# Autodesk Inventor assembly: Tri_Act_lite
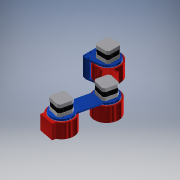
[picture p0: Inventor's stored thumbnail of the model, 180x180]
Saved by Autodesk Inventor 2017 (Build 210142000, 142)
## iProperties
Created: 2019-06-27
Part Number: Tri_Act_lite
Document SubType Name: Assembly
Designer: paulg
Author: paulg
## Documents named in this file (16)
- C:\play\3D_play\Cycloid CAD\Tri_Act_lite.iam
- C:\play\3D_play\Cycloid CAD\Main_equation_hr_big_6810.ipt
- C:\play\3D_play\Cycloid CAD\eq_Outer_tri_body_6810.ipt
- C:\play\3D_play\Cycloid CAD\65x50x7 bearing.ipt
- C:\play\3D_play\robot arm\tri_ecc_cam.ipt
- C:\play\3D_play\Cycloid CAD\Main_equation_hr_big_centre_6810.ipt
- C:\play\3D_play\Cycloid CAD\tri_base_6810.ipt
- C:\play\3D_play\robot arm\Motor_paso.ipt
- C:\play\3D_play\Cycloid CAD\tri_base_free_6810.ipt
- C:\play\3D_play\robot arm\18x12x4 bearing.ipt
- C:\play\3D_play\robot arm\tri_sholder_top_base_lite_part_A.ipt
- C:\play\3D_play\Cycloid CAD\tri_fore_arm_step_6810.ipt
- C:\play\3D_play\Cycloid CAD\eq_Outer_tri_body_end_6810.ipt
- C:\play\3D_play\robot arm\27x20x4 bearing.ipt
- C:\play\3D_play\robot arm\8x5x2.5 bearing.ipt
- C:\play\3D_play\robot arm\inner_rods_44mm.ipt
## Components (36 placed, 15 different names)
1. Main_equation_hr_big_6810:1 — Mate:1, Insert:23
2. eq_Outer_tri_body_6810:1 — Mate:4, Flush:2, Flush:3, Insert:25
3. 65x50x7 bearing:1 — Insert:3, Insert:12
4. 65x50x7 bearing:2 — Insert:10, Insert:25
5. tri_ecc_cam:1 — Insert:3, Insert:5, Insert:13, Insert:23, Insert:24
6. Main_equation_hr_big_6810:2 — Insert:5, Mate:1, Insert:27, Insert:28, Insert:29, Insert:30, Insert:31, Insert:32, Insert:33, Insert:34, Insert:35
7. Main_equation_hr_big_centre_6810:1 — Insert:24
8. tri_base_6810:1 — Insert:10, Insert:11, Mate:2, Flush:1, Insert:14, Insert:15, Insert:36
9. Motor_paso:1 — Insert:11, Mate:2
10. tri_base_free_6810:1 — Insert:12, Flush:1
11. 18x12x4 bearing:1 — Insert:13
12. tri_sholder_top_base_lite_part_A:1 — Insert:14, Insert:15
13. eq_Outer_tri_body_6810:2 — Mate:4, Flush:2, Flush:3, Insert:26
14. 65x50x7 bearing:3 — Insert:26
15. tri_fore_arm_step_6810:1 — Insert:20, Insert:21, Mate:5
16. Motor_paso:2
17. eq_Outer_tri_body_end_6810:1
18. 65x50x7 bearing:4 — Insert:20
19. Motor_paso:3 — Insert:21, Mate:5
20. 27x20x4 bearing:1 — Insert:27
21. 8x5x2.5 bearing:1 — Insert:28
22. 8x5x2.5 bearing:2 — Insert:30
23. 8x5x2.5 bearing:3 — Insert:33
24. 8x5x2.5 bearing:4 — Insert:32
25. 8x5x2.5 bearing:5 — Insert:31
26. 8x5x2.5 bearing:6 — Insert:29
27. 8x5x2.5 bearing:7 — Insert:35
28. 8x5x2.5 bearing:8 — Insert:34
29. inner_rods_44mm:1 — Insert:36
30. inner_rods_44mm:2
31. inner_rods_44mm:3
32. inner_rods_44mm:4
33. inner_rods_44mm:5
34. inner_rods_44mm:6
35. inner_rods_44mm:7
36. inner_rods_44mm:8
## Component patterns: (8 elements, first: inner_rods_44mm:1)
## Relationships (35: Insert 27, Mate 5, Flush 3)
- Insert:3: 65x50x7 bearing:1 ↔ tri_ecc_cam:1
- Insert:5 (0.5 mm): tri_ecc_cam:1 ↔ Main_equation_hr_big_6810:2
- Mate:1: Main_equation_hr_big_6810:1 ↔ Main_equation_hr_big_6810:2
- Insert:10: 65x50x7 bearing:2 ↔ tri_base_6810:1
- Insert:11: tri_base_6810:1 ↔ Motor_paso:1
- Mate:2: tri_base_6810:1 ↔ Motor_paso:1
- Insert:12: 65x50x7 bearing:1 ↔ tri_base_free_6810:1
- Flush:1: tri_base_6810:1 ↔ tri_base_free_6810:1
- Insert:13: tri_ecc_cam:1 ↔ 18x12x4 bearing:1
- Insert:14: tri_base_6810:1 ↔ tri_sholder_top_base_lite_part_A:1
- Insert:15: tri_base_6810:1 ↔ tri_sholder_top_base_lite_part_A:1
- [Insert]: 65x50x7 bearing:3 ↔ tri_fore_arm_step_6810:1
- [Insert]: tri_fore_arm_step_6810:1 ↔ Motor_paso:2
- [Mate]: tri_fore_arm_step_6810:1 ↔ Motor_paso:2
- Mate:4: eq_Outer_tri_body_6810:1 ↔ eq_Outer_tri_body_6810:2
- [Insert]: eq_Outer_tri_body_end_6810:1 ↔ 65x50x7 bearing:4
- Insert:20: tri_fore_arm_step_6810:1 ↔ 65x50x7 bearing:4
- Insert:21: tri_fore_arm_step_6810:1 ↔ Motor_paso:3
- Mate:5: tri_fore_arm_step_6810:1 ↔ Motor_paso:3
- Flush:2: eq_Outer_tri_body_6810:1 ↔ eq_Outer_tri_body_6810:2
- Flush:3: eq_Outer_tri_body_6810:1 ↔ eq_Outer_tri_body_6810:2
- Insert:23: Main_equation_hr_big_6810:1 ↔ tri_ecc_cam:1
- Insert:24 (-5 mm): tri_ecc_cam:1 ↔ Main_equation_hr_big_centre_6810:1
- Insert:25: eq_Outer_tri_body_6810:1 ↔ 65x50x7 bearing:2
- Insert:26: eq_Outer_tri_body_6810:2 ↔ 65x50x7 bearing:3
- Insert:27: Main_equation_hr_big_6810:2 ↔ 27x20x4 bearing:1
- Insert:28: Main_equation_hr_big_6810:2 ↔ 8x5x2.5 bearing:1
- Insert:29: Main_equation_hr_big_6810:2 ↔ 8x5x2.5 bearing:6
- Insert:30: Main_equation_hr_big_6810:2 ↔ 8x5x2.5 bearing:2
- Insert:31: Main_equation_hr_big_6810:2 ↔ 8x5x2.5 bearing:5
- Insert:32: Main_equation_hr_big_6810:2 ↔ 8x5x2.5 bearing:4
- Insert:33: Main_equation_hr_big_6810:2 ↔ 8x5x2.5 bearing:3
- Insert:34: Main_equation_hr_big_6810:2 ↔ 8x5x2.5 bearing:8
- Insert:35: Main_equation_hr_big_6810:2 ↔ 8x5x2.5 bearing:7
- Insert:36: tri_base_6810:1 ↔ inner_rods_44mm:1
## Named parameters: d19_d12 = 0 mm, d20_d13 = 0 mm, d21_d11 = 0 mm, d29_d22_d1 = 0 mm
